# Autodesk Inventor assembly: Cube 1x1 V5 (One Inch Lense)
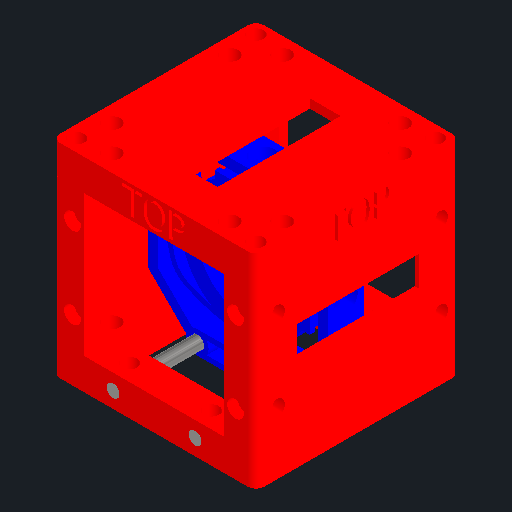
[picture p0: Inventor's stored thumbnail of the model, 512x512]
Saved by Autodesk Inventor 2023.4 (Build 274418000, 418)
## iProperties
Created: 2022-08-13
Part Number: Cube 1x1 V5 (One Inch Lense)
Document SubType Name: Assembly
Designer: xSibe
Author: xSibe
## Documents named in this file (5)
- C:\.Laptop\.Work\Projects\Project Protocube\Protocube\CAD, STL, OBJ Files\1 CAD\Lense\Cube 1x1 V5 (One Inch Lense).iam
- C:\.Laptop\.Work\Projects\Project Protocube\Protocube\CAD, STL, OBJ Files\1 CAD\Attachments\Mounting Bar.ipt
- C:\.Laptop\.Work\Projects\Project Protocube\Protocube\CAD, STL, OBJ Files\1 CAD\Lense\One Inch Lense Holder (V5).ipt
- C:\.Laptop\.Work\Projects\Project Protocube\Protocube\CAD, STL, OBJ Files\1 CAD\Cubes\Cube 1x1 V5 Closed Slotted.iam
- C:\.Laptop\.Work\Projects\Project Protocube\Protocube\CAD, STL, OBJ Files\1 CAD\Lense\One Inch Lense Holder Cover (V5).ipt
## Components (4 placed, 4 different names)
1. Mounting Bar:1
2. One Inch Lense Holder (V5):1 — Mate:1, Mate:2
3. Cube 1x1 V5 Closed Slotted:1 [sub-assembly]
4. One Inch Lense Holder Cover (V5):1 — Mate:1, Mate:2, Flush:1
## Relationships (3: Mate 2, Flush 1)
- Mate:1: One Inch Lense Holder (V5):1 ↔ One Inch Lense Holder Cover (V5):1
- Mate:2: One Inch Lense Holder (V5):1 ↔ One Inch Lense Holder Cover (V5):1
- Flush:1: One Inch Lense Holder Cover (V5):1
